# Autodesk Inventor assembly: Verpackung
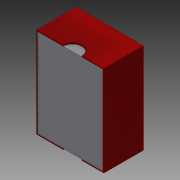
[picture p0: Inventor's stored thumbnail of the model, 180x180]
Saved by Autodesk Inventor 2014 (Build 180170000, 170)
## iProperties
Created: 2016-09-06
Part Number: Verpackung
Document SubType Name: Assembly
Designer: cem
Author: cem
## Documents named in this file (5)
- C:\development\AnySense\Hardware\Verpackung\Verpackung.iam
- C:\development\AnySense\Hardware\Verpackung\Boden.ipt
- C:\development\AnySense\Hardware\Verpackung\InlayUnten.ipt
- C:\development\AnySense\Hardware\Verpackung\InlayOben.ipt
- C:\development\AnySense\Hardware\Verpackung\Deckel.ipt
## Components (4 placed, 4 different names)
1. Boden:1 — Fluchtend:1, Fluchtend:2, Fluchtend:5, Fluchtend:6
2. InlayUnten:1 — Fluchtend:1, Fluchtend:2, Fluchtend:3, Fluchtend:4
3. InlayOben:1 — Fluchtend:3, Fluchtend:4
4. Deckel:1 — Fluchtend:5, Fluchtend:6
## Relationships (6: Flush 6)
- Fluchtend:1 [Flush]: Boden:1 ↔ InlayUnten:1
- Fluchtend:2 [Flush]: Boden:1 ↔ InlayUnten:1
- Fluchtend:3 [Flush]: InlayUnten:1 ↔ InlayOben:1
- Fluchtend:4 [Flush]: InlayUnten:1 ↔ InlayOben:1
- Fluchtend:5 [Flush]: Boden:1 ↔ Deckel:1
- Fluchtend:6 [Flush] (0.5 mm): Boden:1 ↔ Deckel:1
